# Autodesk Inventor assembly: Computer box
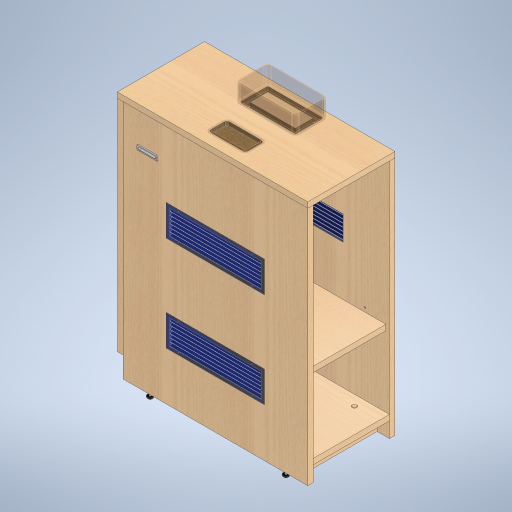
[picture p0: Inventor's stored thumbnail of the model, 512x512]
Saved by Autodesk Inventor 2024 (Build 280153000, 153)
## iProperties
Created: 2021-12-30
Part Number: Computer box
Document SubType Name: Assembly
Designer: sauliusd
Author: sauliusd
## Documents named in this file (19)
- C:\W4INV 2024 Design\PROJECTS\Samples\Macro DEMO\7 Computer Box\Computer box.iam
- C:\W4INV 2024 Design\PROJECTS\Samples\Macro DEMO\7 Computer Box\Left Side.ipt
- C:\W4INV 2024 Design\PROJECTS\Samples\Macro DEMO\7 Computer Box\Top.ipt
- C:\W4INV 2024 Design\PROJECTS\Samples\Macro DEMO\7 Computer Box\Right Side.ipt
- C:\W4INV 2024 Design\PROJECTS\Samples\Macro DEMO\7 Computer Box\Bottom.ipt
- C:\W4INV 2024 Design\PROJECTS\Samples\Macro DEMO\7 Computer Box\Shelf.ipt
- C:\W4INV 2024 Design\PROJECTS\Samples\Macro DEMO\7 Computer Box\Plynth.ipt
- C:\W4INV 2024 Design\PROJECTS\Samples\Macro DEMO\7 Computer Box\Back.ipt
- C:\W4INV 2022 Design\_LIBRARY\Holders\Shelf holder D5\Shelf support D5 L16 with hole covers.ipt
- C:\W4INV 2022 Design\LIBRARY\Holders\Shelf holder D5.ipt
- C:\W4INV 2024 Design\LIBRARY\Fixed joints\Minifix joint\Minifix D15\Minifix D15.iam
- C:\W4INV 2024 Design\LIBRARY\Fixed joints\Confirmat\Confirmat\confirmat.iam
- C:\W4INV 2024 Design\PROJECTS\Samples\Macro DEMO\4 Ventilation Grill\Ventilation Grille.ipt
- C:\W4INV 2024 Design\PROJECTS\Samples\Macro DEMO\3 Alternate Side processing definition\Aisle.ipt
- C:\W4INV 2024 Design\_LIBRARY\Supports and legs\Supports\ADJUSTABLE SUPPORT\Support M6 H27 D18 with Bushing SB T18.ipt
- C:\W4INV 2022 Design\LIBRARY\Supports and legs\Supports\ADJUSTABLE SUPPORT.ipt
- C:\W4INV 2024 Design\PROJECTS\Samples\Macro DEMO\5 Lamello Clamex P-14\Clamex P-14 Connector.iam
- C:\W4INV 2024 Design\PROJECTS\Samples\Macro DEMO\1 Parameter Usage\Holder for paper clips.ipt
- C:\W4INV 2024 Design\PROJECTS\Samples\Macro DEMO\2 Ways of Macro rotation definition\Table top pencil case.ipt
## Components (41 placed, 16 different names)
1. Left Side:1 — Flush:1, Flush:2, Side Board Plane:1, Side Board Plane:3, Nestled Plate:7, Nestled Plate:9, Surface for Insertion:1, Surface for Insertion:3, Main Plane:3, Side board:1, Bottom board:1, Bottom board:2, Side board:3, Bottom board:3, Bottom board:4, Joining Plane Solution 1:1, Edge or Inner Plane:1, Joining Plane Solution 1:2, Edge or Inner Plane:2, Joining Plane Solution 1:3, Edge or Inner Plane:3, Pillar_Board_Plane:2, Pillar_Board_Plane:4
2. Top:1 — Align To Edge Plane:5, Align To Edge Plane:6, Desktop Plane:1, Orientation:1, Table Top:1
3. Right Side:1 — Side Board Plane:2, Side Board Plane:4, Nestled Plate:8, Nestled Plate:10, Surface for Insertion:2, Surface for Insertion:4, Main Plane:4, Side board:2, Side board:4, Joining Plane Solution 1:4, Edge or Inner Plane:4, Joining Plane Solution 1:5, Edge or Inner Plane:5, Joining Plane Solution 1:6, Edge or Inner Plane:6, Pillar_Board_Plane:1, Pillar_Board_Plane:3
4. Bottom:1 — Flush:4, Pillar Plate:7, Pillar Plate:8, Pillar Plate:9, Pillar Plate:10
5. Shelf:1 — Flush:3, Shelf Pottom Plane:1, Shelf Pottom Plane:2, Shelf Pottom Plane:3, Shelf Pottom Plane:4
6. Plynth:1
7. Back:1 — Surface for Insertion:5, Axis Plane 1:5, Surface for Insertion:6, Axis Plane 1:6, Main Plane:1, Second Axis:1, Main Plane:2, Second Axis:2, Axis_Plane:1, Nestled_Board_Plane:1, Axis_Plane:2, Nestled_Board_Plane:2, Axis_Plane:3, Nestled_Board_Plane:3, Axis_Plane:4, Nestled_Board_Plane:4, Second Axis:5, Orientation Axis:1
8. Shelf support D5 L16 with hole covers:1 — Axis Plane:1, Side Board Plane:1, Shelf Pottom Plane:1
9. Shelf support D5 L16 with hole covers:2 — Axis Plane:2, Side Board Plane:2, Shelf Pottom Plane:2
10. Shelf support D5 L16 with hole covers:3 — Axis Plane:3, Side Board Plane:3, Shelf Pottom Plane:3
11. Shelf support D5 L16 with hole covers:4 — Axis Plane:4, Side Board Plane:4, Shelf Pottom Plane:4
12. Minifix D15:7 [sub-assembly] — Center Axis:7, Nestled Plate:7, Pillar Plate:7
13. Minifix D15:8 [sub-assembly] — Center Axis:8, Nestled Plate:8, Pillar Plate:8
14. Minifix D15:9 [sub-assembly] — Center Axis:9, Nestled Plate:9, Pillar Plate:9
15. Minifix D15:10 [sub-assembly] — Center Axis:10, Nestled Plate:10, Pillar Plate:10
16. Ventilation Grille:2 — Axis Plane 1:1, Surface for Insertion:1, Axis Plane 2:1, Align To Edge Plane:1
17. Ventilation Grille:3 — Axis Plane 1:2, Surface for Insertion:2, Axis Plane 2:2, Align To Edge Plane:2
18. Ventilation Grille:4 — Axis Plane 1:3, Surface for Insertion:3, Axis Plane 2:3, Align To Edge Plane:3
19. Ventilation Grille:5 — Axis Plane 1:4, Surface for Insertion:4, Axis Plane 2:4, Align To Edge Plane:4
20. Ventilation Grille:6 — Axis Plane 2:5, Surface for Insertion:5, Axis Plane 1:5, Align To Edge Plane:5
21. Ventilation Grille:7 — Axis Plane 2:6, Surface for Insertion:6, Axis Plane 1:6, Align To Edge Plane:6
22. Aisle:1 — Main Plane:1, Orientation Plane:1, Second Axis:1
23. Aisle:2 — Main Plane:2, Orientation Plane:2, Second Axis:2
24. Aisle:3 — Main Plane:3, Orientation Plane:3, Second Axis:3
25. Aisle:4 — Main Plane:4, Orientation Plane:4, Second Axis:4
26. Support M6 H27 D18 with Bushing SB T18:3 — Axis:1, Side board:1, Bottom board:1
27. Support M6 H27 D18 with Bushing SB T18:4 — Axis:2, Side board:2, Bottom board:2
28. Support M6 H27 D18 with Bushing SB T18:5 — Axis:3, Side board:3, Bottom board:3
29. Support M6 H27 D18 with Bushing SB T18:6 — Axis:4, Side board:4, Bottom board:4
30. Clamex P-14 Connector:2 [sub-assembly] — Joining Plane Solution 1:1, Edge or Inner Plane:1, Center Point Match Plane:1
31. Clamex P-14 Connector:3 [sub-assembly] — Joining Plane Solution 1:2, Edge or Inner Plane:2, Center Point Match Plane:2
32. Clamex P-14 Connector:4 [sub-assembly] — Joining Plane Solution 1:3, Edge or Inner Plane:3, Center Point Match Plane:3
33. Clamex P-14 Connector:5 [sub-assembly] — Joining Plane Solution 1:4, Edge or Inner Plane:4, Center Point Match Plane:4
34. Clamex P-14 Connector:6 [sub-assembly] — Center Point Match Plane:5, Joining Plane Solution 1:5, Edge or Inner Plane:5
35. Clamex P-14 Connector:7 [sub-assembly] — Center Point Match Plane:6, Joining Plane Solution 1:6, Edge or Inner Plane:6
36. confirmat:1 [sub-assembly] — Axis_Plane:1, Pillar_Board_Plane:1, Nestled_Board_Plane:1
37. confirmat:2 [sub-assembly] — Axis_Plane:2, Pillar_Board_Plane:2, Nestled_Board_Plane:2
38. confirmat:3 [sub-assembly] — Axis_Plane:3, Pillar_Board_Plane:3, Nestled_Board_Plane:3
39. confirmat:4 [sub-assembly] — Axis_Plane:4, Pillar_Board_Plane:4, Nestled_Board_Plane:4
40. Holder for paper clips:1 — Desktop Plane:1, First Axis:1, Second Axis:5, Orientation:1
41. Table top pencil case:1 — Table Top:1, Orientation Axis:1, Second Axis:6
## Relationships (117: Mate 72, Flush 37, Angle 7, Symmetry 1)
- Flush:1 (-80 mm): Left Side:1
- Flush:2 (-98 mm): Left Side:1
- Flush:3 (200 mm): Shelf:1
- Flush:4 (140 mm): Bottom:1
- Axis Plane:1 [Mate]: Shelf support D5 L16 with hole covers:1
- Side Board Plane:1 [Mate]: Left Side:1 ↔ Shelf support D5 L16 with hole covers:1
- Shelf Pottom Plane:1 [Mate] (2.5 mm): Shelf:1 ↔ Shelf support D5 L16 with hole covers:1
- Axis Plane:2 [Mate]: Shelf support D5 L16 with hole covers:2
- Side Board Plane:2 [Mate]: Right Side:1 ↔ Shelf support D5 L16 with hole covers:2
- Shelf Pottom Plane:2 [Mate] (2.5 mm): Shelf:1 ↔ Shelf support D5 L16 with hole covers:2
- Axis Plane:3 [Mate]: Shelf support D5 L16 with hole covers:3
- Side Board Plane:3 [Mate]: Left Side:1 ↔ Shelf support D5 L16 with hole covers:3
- Shelf Pottom Plane:3 [Mate] (2.5 mm): Shelf:1 ↔ Shelf support D5 L16 with hole covers:3
- Axis Plane:4 [Mate]: Shelf support D5 L16 with hole covers:4
- Side Board Plane:4 [Mate]: Right Side:1 ↔ Shelf support D5 L16 with hole covers:4
- Shelf Pottom Plane:4 [Mate] (2.5 mm): Shelf:1 ↔ Shelf support D5 L16 with hole covers:4
- Center Axis:7 [Mate]: Minifix D15:7
- Nestled Plate:7 [Mate]: Left Side:1 ↔ Minifix D15:7
- Pillar Plate:7 [Flush]: Bottom:1 ↔ Minifix D15:7
- Center Axis:8 [Mate]: Minifix D15:8
- Nestled Plate:8 [Mate]: Right Side:1 ↔ Minifix D15:8
- Pillar Plate:8 [Flush]: Bottom:1 ↔ Minifix D15:8
- Center Axis:9 [Mate]: Minifix D15:9
- Nestled Plate:9 [Mate]: Left Side:1 ↔ Minifix D15:9
- Pillar Plate:9 [Flush]: Bottom:1 ↔ Minifix D15:9
- Center Axis:10 [Mate]: Minifix D15:10
- Nestled Plate:10 [Mate]: Right Side:1 ↔ Minifix D15:10
- Pillar Plate:10 [Flush]: Bottom:1 ↔ Minifix D15:10
- Symmetry:1
- Axis Plane 1:1 [Mate]: Ventilation Grille:2
- Surface for Insertion:1 [Flush]: Left Side:1 ↔ Ventilation Grille:2
- Axis Plane 2:1 [Mate]: Ventilation Grille:2
- Align To Edge Plane:1 [Angle] (0 deg): Ventilation Grille:2
- Axis Plane 1:2 [Mate]: Ventilation Grille:3
- Surface for Insertion:2 [Flush]: Right Side:1 ↔ Ventilation Grille:3
- Axis Plane 2:2 [Mate]: Ventilation Grille:3
- Align To Edge Plane:2 [Angle] (0 deg): Ventilation Grille:3
- Axis Plane 1:3 [Mate]: Ventilation Grille:4
- Surface for Insertion:3 [Flush]: Left Side:1 ↔ Ventilation Grille:4
- Axis Plane 2:3 [Mate]: Ventilation Grille:4
- Align To Edge Plane:3 [Angle] (0 deg): Ventilation Grille:4
- Axis Plane 1:4 [Mate]: Ventilation Grille:5
- Surface for Insertion:4 [Flush]: Right Side:1 ↔ Ventilation Grille:5
- Axis Plane 2:4 [Mate]: Ventilation Grille:5
- Align To Edge Plane:4 [Angle] (0 deg): Ventilation Grille:5
- Axis Plane 2:5 [Mate]: Ventilation Grille:6
- Surface for Insertion:5 [Flush]: Back:1 ↔ Ventilation Grille:6
- Axis Plane 1:5 [Mate]: Back:1 ↔ Ventilation Grille:6
- Align To Edge Plane:5 [Angle] (0 deg): Top:1 ↔ Ventilation Grille:6
- Axis Plane 2:6 [Mate]: Ventilation Grille:7
- Surface for Insertion:6 [Flush]: Back:1 ↔ Ventilation Grille:7
- Axis Plane 1:6 [Mate]: Back:1 ↔ Ventilation Grille:7
- Align To Edge Plane:6 [Angle] (0 deg): Top:1 ↔ Ventilation Grille:7
- Flush:23 (160 mm)
- Flush:24 (-120 mm)
- Flush:25 (-80 mm)
- Main Plane:1 [Mate]: Back:1 ↔ Aisle:1
- Orientation Plane:1 [Flush]: Aisle:1
- Second Axis:1 [Mate]: Back:1 ↔ Aisle:1
- Main Plane:2 [Mate]: Back:1 ↔ Aisle:2
- Orientation Plane:2 [Flush]: Aisle:2
- Second Axis:2 [Mate]: Back:1 ↔ Aisle:2
- Main Plane:3 [Mate]: Left Side:1 ↔ Aisle:3
- Orientation Plane:3 [Flush]: Aisle:3
- Second Axis:3 [Mate]: Aisle:3
- Main Plane:4 [Mate]: Right Side:1 ↔ Aisle:4
- Orientation Plane:4 [Flush]: Aisle:4
- Second Axis:4 [Mate]: Aisle:4
- Axis:1 [Mate]: Support M6 H27 D18 with Bushing SB T18:3
- Side board:1 [Flush] (9 mm): Left Side:1 ↔ Support M6 H27 D18 with Bushing SB T18:3
- Bottom board:1 [Mate] (17.5 mm): Left Side:1 ↔ Support M6 H27 D18 with Bushing SB T18:3
- Axis:2 [Mate]: Support M6 H27 D18 with Bushing SB T18:4
- Side board:2 [Flush] (9 mm): Right Side:1 ↔ Support M6 H27 D18 with Bushing SB T18:4
- Bottom board:2 [Mate] (17.5 mm): Left Side:1 ↔ Support M6 H27 D18 with Bushing SB T18:4
- Axis:3 [Mate]: Support M6 H27 D18 with Bushing SB T18:5
- Side board:3 [Flush] (9 mm): Left Side:1 ↔ Support M6 H27 D18 with Bushing SB T18:5
- Bottom board:3 [Mate] (17.5 mm): Left Side:1 ↔ Support M6 H27 D18 with Bushing SB T18:5
- Axis:4 [Mate]: Support M6 H27 D18 with Bushing SB T18:6
- Side board:4 [Flush] (9 mm): Right Side:1 ↔ Support M6 H27 D18 with Bushing SB T18:6
- Bottom board:4 [Mate] (17.5 mm): Left Side:1 ↔ Support M6 H27 D18 with Bushing SB T18:6
- Joining Plane Solution 1:1 [Flush]: Left Side:1 ↔ Clamex P-14 Connector:2
- Edge or Inner Plane:1 [Mate]: Left Side:1 ↔ Clamex P-14 Connector:2
- Center Point Match Plane:1 [Mate]: Clamex P-14 Connector:2
- Joining Plane Solution 1:2 [Flush]: Left Side:1 ↔ Clamex P-14 Connector:3
- Edge or Inner Plane:2 [Mate]: Left Side:1 ↔ Clamex P-14 Connector:3
- Center Point Match Plane:2 [Mate]: Clamex P-14 Connector:3
- Joining Plane Solution 1:3 [Flush]: Left Side:1 ↔ Clamex P-14 Connector:4
- Edge or Inner Plane:3 [Mate]: Left Side:1 ↔ Clamex P-14 Connector:4
- Center Point Match Plane:3 [Mate]: Clamex P-14 Connector:4
- Joining Plane Solution 1:4 [Flush]: Right Side:1 ↔ Clamex P-14 Connector:5
- Edge or Inner Plane:4 [Mate]: Right Side:1 ↔ Clamex P-14 Connector:5
- Center Point Match Plane:4 [Mate]: Clamex P-14 Connector:5
- Center Point Match Plane:5 [Mate]: Clamex P-14 Connector:6
- Joining Plane Solution 1:5 [Flush]: Right Side:1 ↔ Clamex P-14 Connector:6
- Edge or Inner Plane:5 [Mate]: Right Side:1 ↔ Clamex P-14 Connector:6
- Center Point Match Plane:6 [Mate]: Clamex P-14 Connector:7
- Joining Plane Solution 1:6 [Flush]: Right Side:1 ↔ Clamex P-14 Connector:7
- Edge or Inner Plane:6 [Mate]: Right Side:1 ↔ Clamex P-14 Connector:7
- Axis_Plane:1 [Mate]: Back:1 ↔ confirmat:1
- Pillar_Board_Plane:1 [Mate] (-9 mm): Right Side:1 ↔ confirmat:1
- Nestled_Board_Plane:1 [Flush]: Back:1 ↔ confirmat:1
- Axis_Plane:2 [Mate]: Back:1 ↔ confirmat:2
- Pillar_Board_Plane:2 [Mate] (-9 mm): Left Side:1 ↔ confirmat:2
- Nestled_Board_Plane:2 [Flush]: Back:1 ↔ confirmat:2
- Axis_Plane:3 [Mate]: Back:1 ↔ confirmat:3
- Pillar_Board_Plane:3 [Mate] (-9 mm): Right Side:1 ↔ confirmat:3
- Nestled_Board_Plane:3 [Flush]: Back:1 ↔ confirmat:3
- Axis_Plane:4 [Mate]: Back:1 ↔ confirmat:4
- Pillar_Board_Plane:4 [Mate] (-9 mm): Left Side:1 ↔ confirmat:4
- Nestled_Board_Plane:4 [Flush]: Back:1 ↔ confirmat:4
- Desktop Plane:1 [Mate]: Top:1 ↔ Holder for paper clips:1
- First Axis:1 [Mate]: Holder for paper clips:1
- Second Axis:5 [Mate]: Back:1 ↔ Holder for paper clips:1
- Orientation:1 [Angle] (0 deg): Top:1 ↔ Holder for paper clips:1
- Table Top:1 [Flush]: Top:1 ↔ Table top pencil case:1
- Orientation Axis:1 [Flush]: Back:1 ↔ Table top pencil case:1
- Second Axis:6 [Mate]: Table top pencil case:1
